# Autodesk Inventor assembly: Rolling Joint
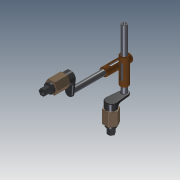
[picture p0: Inventor's stored thumbnail of the model, 180x180]
Saved by Autodesk Inventor 2015 (Build 190159000, 159)
## iProperties
Created: 2021-03-29
Part Number: Rolling Joint
Document SubType Name: Assembly
Designer: Diptanshu Das
Author: Diptanshu Das
## Documents named in this file (4)
- D:\Entraco_workspace\3D\Animation\Rolling Joint\Rolling Joint\Rolling Joint.iam
- D:\Entraco_workspace\3D\Animation\Rolling Joint\Rolling Joint\Arm.ipt
- D:\Entraco_workspace\3D\Animation\Rolling Joint\Rolling Joint\Nut.ipt
- D:\Entraco_workspace\3D\Animation\Rolling Joint\Rolling Joint\Socket.ipt
## Components (5 placed, 3 different names)
1. Arm:1 — Mate:1, Mate:2, Mate:3, Mate:4, Mate:6, Angle:1, Rotation:1
2. Nut:1 — Mate:3, Mate:4, Mate:5
3. Socket:1 — Mate:6, Mate:13
4. Arm:2 — Flush:1, Mate:12, Mate:13, Mate:14, Mate:15, Rotation:1
5. Nut:2 — Mate:14, Mate:15, Mate:16
## Relationships (17: Mate 13, Flush 2, Angle 1, RelateRotation 1)
- Mate:1: Arm:1
- Mate:2: Arm:1
- Mate:3: Arm:1 ↔ Nut:1
- Mate:4: Arm:1 ↔ Nut:1
- Mate:5: Nut:1
- Mate:6: Arm:1 ↔ Socket:1
- Flush:1 (250 mm): Arm:2
- Flush:2 (265 mm)
- Mate:10
- Mate:11 (60 mm)
- Mate:12: Arm:2
- Mate:13: Socket:1 ↔ Arm:2
- Mate:14: Arm:2 ↔ Nut:2
- Mate:15: Arm:2 ↔ Nut:2
- Mate:16: Nut:2
- Angle:1 (0 deg): Arm:1
- Rotation:1 [RelateRotation] (1 ul): Arm:1 ↔ Arm:2
